(part 1 of 2)
# Autodesk Inventor assembly: #SHOOTER.3
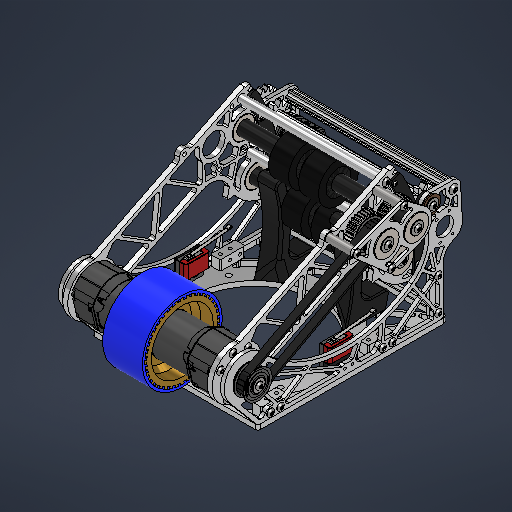
[picture p0: Inventor's stored thumbnail of the model, 512x512]
Saved by Autodesk Inventor 2026.1 (Build 301233020, 233B)
## iProperties
Created: 2026-01-27
Part Number: #SHOOTER.3
Document SubType Name: Assembly
Designer: Owen L
Mass: 5560.26 g
Surface Area: 8956.44 cm^2
Volume: 1678.59 cm^3
Density: 3.31246 g/cm^3
Author: Owen L
## Documents named in this file (55)
- C:\Users\Owen\Documents\GitHub\2026-Robot-Mechanical\Shooter\Shooter - Front Motors\#SHOOTER.FRONT_MOTORS.iam
- C:\Users\Owen\Documents\GitHub\2026-Robot-Mechanical\Shooter\Shooter - Front Motors\PLATE,SHOOTER,SIDE.ipt
- C:\Users\Owen\Documents\GitHub\2026-Robot-Mechanical\#1_CAD Library\Electronics\CONTROLS,SPARK_FLEX.ipt
- C:\Users\Owen\Documents\GitHub\2026-Robot-Mechanical\#1_CAD Library\Power Transmission\Bushings\PURCHASED,BUSHING,13.75mmID,0.75inOD.ipt
- C:\Users\Owen\Documents\GitHub\2026-Robot-Mechanical\#1_CAD Library\Power Transmission\Bearings\PURCHASED,HEX_BEARING.ipt
- C:\Users\Owen\Documents\GitHub\2026-Robot-Mechanical\#1_CAD Library\Motors\MOTOR,REV,NEO,VORTEX.ipt
- C:\Users\Owen\Documents\GitHub\2026-Robot-Mechanical\#1_CAD Library\Motors\MOTOR,REV,NEO,550.ipt
- C:\Users\Owen\Documents\GitHub\2026-Robot-Mechanical\#1_CAD Library\Power Transmission\UltraPlanetary\PURCHASED,REV,ULTRAPLANETARY,2-STAGE.iam
- C:\Users\Owen\Documents\GitHub\2026-Robot-Mechanical\Shooter\Shooter - Front Motors\#SHOOTER.3\Design Accelerator\PLATE,HOOD,SIDE.ipt
- C:\Users\Owen\Documents\GitHub\2026-Robot-Mechanical\Shooter\Shooter - Front Motors\#SHOOTER.3\Design Accelerator\PLATE.HOOD,PINION,GEAR.ipt
- C:\Users\Owen\Documents\GitHub\2026-Robot-Mechanical\Shooter\Shooter - Front Motors\STOCK,HEX,ROUND,HOOD.ipt
- C:\Users\Owen\Documents\GitHub\2026-Robot-Mechanical\#1_CAD Library\Power Transmission\Pulleys\PURCHASED,HTD5mm,20T,PULLEY.ipt
- C:\Users\Owen\Documents\GitHub\2026-Robot-Mechanical\Shooter\Shooter - Front Motors\#SHOOTER.3\Design Accelerator\PLATE,HOOD,DRIVE,GEAR,SHAFT.ipt
- C:\Users\Owen\Documents\GitHub\2026-Robot-Mechanical\Shooter\Shooter - Front Motors\#SHOOTER.3\Design Accelerator\PLATE,HOOD,DRIVE,GEAR,MOTOR.ipt
- C:\Users\Owen\Documents\GitHub\2026-Robot-Mechanical\Shooter\Shooter - Front Motors\STOCK,SHAFT,HEX,SHOOTER.ipt
- C:\Users\Owen\Documents\GitHub\2026-Robot-Mechanical\Shooter\Shooter - Front Motors\#SHOOTER.3\PURCHASED,10-32,0.375inOD,STANDOFF.ipt
- C:\Users\Owen\Documents\GitHub\2026-Robot-Mechanical\Shooter\Shooter - Front Motors\PLATE,BEARING,MOUNT.ipt
- C:\Users\Owen\Documents\GitHub\2026-Robot-Mechanical\Shooter\Shooter - Front Motors\STOCK,SHAFT,HEX,HOOD,WHEELS,LONG.ipt
- C:\Users\Owen\Documents\GitHub\2026-Robot-Mechanical\Shooter\Shooter - Front Motors\STOCK,SHAFT,HEX,HOOD,REVERSER.ipt
- C:\Users\Owen\Documents\GitHub\2026-Robot-Mechanical\Shooter\Shooter - Front Motors\STOCK,SHAFT,HEX,HOOD,WHEELS,SHORT.ipt
- C:\Users\Owen\Documents\GitHub\2026-Robot-Mechanical\Shooter\Shooter - Front Motors\PLATE,SHOOTER,BOTTOM.ipt
- C:\Users\Owen\Documents\GitHub\2026-Robot-Mechanical\Shooter\Shooter - Front Motors\PLATE,SHOOTER,BACK.ipt
- C:\Users\Owen\Documents\GitHub\2026-Robot-Mechanical\Shooter\Shooter - Front Motors\STOCK,CHURRO,HEX,BACK.ipt
- C:\Users\Owen\Documents\GitHub\2026-Robot-Mechanical\Shooter\Shooter - Front Motors\PURCHASED,WASHER.ipt
- C:\Users\Owen\Documents\GitHub\2026-Robot-Mechanical\#1_CAD Library\Wheels\Shooter\PURCHASED,2inOD,HEX,SHOOTER,WHEEL.ipt
- C:\Users\Owen\Documents\GitHub\2026-Robot-Mechanical\#1_CAD Library\Building Materials\Fasteners\Bolts\PURCHASED,0.25-20x0.5in,BUTTONHEAD,BOLT.ipt
- C:\Users\Owen\Documents\GitHub\2026-Robot-Mechanical\#1_CAD Library\Building Materials\Fasteners\Bolts\PURCHASED,10-32x0.5in,BUTTONHEAD,BOLT.ipt
- C:\Users\Owen\Documents\GitHub\2026-Robot-Mechanical\#1_CAD Library\Building Materials\Fasteners\Bolts\PURCHASED,M3x10mm,BUTTONHEAD,BOLT.ipt
- C:\Users\Owen\Documents\GitHub\2026-Robot-Mechanical\Shooter\Shooter - Front Motors\3DPRINT,HOOD,DRIVEGEAR,SPACER.ipt
- C:\Users\Owen\Documents\GitHub\2026-Robot-Mechanical\Shooter\Shooter - Front Motors\3DPRINT,REVERSERGEAR,SPACER.ipt
- C:\Users\Owen\Documents\GitHub\2026-Robot-Mechanical\Shooter\Shooter - Front Motors\3DPRINT,BACKROLLERS,OPENSIDE,SPACER.ipt
- C:\Users\Owen\Documents\GitHub\2026-Robot-Mechanical\Shooter\Shooter - Front Motors\3DPRINT,BACKROLLERS,PULLEYSIDE,SPACER.ipt
- C:\Users\Owen\Documents\GitHub\2026-Robot-Mechanical\Shooter\Shooter - Front Motors\3DPRINT,BACKROLLERS,INTERROLLER,SPACER.ipt
- C:\Users\Owen\Documents\GitHub\2026-Robot-Mechanical\#1_CAD Library\Power Transmission\Gears\PURCHASED,GEAR,20DP,30T,HEX.ipt
- C:\Users\Owen\Documents\GitHub\2026-Robot-Mechanical\Shooter\Shooter - Front Motors\3DPRINT,BACKRAIL.ipt
- C:\Users\Owen\Documents\GitHub\2026-Robot-Mechanical\Shooter\Shooter - Front Motors\3DPRINT,BACKRAIL_MIR.ipt
- C:\Users\Owen\Documents\GitHub\2026-Robot-Mechanical\Shooter\Shooter - Front Motors\PLATE,NUTBLOCK.ipt
- C:\Users\Owen\Documents\GitHub\2026-Robot-Mechanical\#1_CAD Library\Building Materials\Fasteners\Bolts\PURCHASED,M4x12mm,BUTTONHEAD,BOLT.ipt
- C:\Users\Owen\Documents\GitHub\2026-Robot-Mechanical\Shooter\Shooter - Front Motors\STANDIN,45T,HTD5mm,BELT.ipt
- C:\Users\Owen\Documents\GitHub\2026-Robot-Mechanical\Shooter\Shooter - Front Motors\STANDIN,90T,HTD5mm,BELT.ipt
- C:\Users\Owen\Documents\GitHub\2026-Robot-Mechanical\Shooter\Shooter - Front Motors\3DPRINT,FLYWHEELTOHOOD,SPACER.ipt
- C:\Users\Owen\Documents\GitHub\2026-Robot-Mechanical\Shooter\Shooter - Front Motors\STOCK,HOOD,SPACER,10-32,6.25in.ipt
- C:\Users\Owen\Documents\GitHub\2026-Robot-Mechanical\Shooter\Shooter - Front Motors\3DPRINT,SIDEPLATETOHOOD,SPACER .ipt
- C:\Users\Owen\Documents\GitHub\2026-Robot-Mechanical\Shooter\Shooter - Front Motors\3DPRINT,SIDEPLATETOHOODGEAR,SPACER.ipt
- C:\Users\Owen\Documents\GitHub\2026-Robot-Mechanical\Shooter\Shooter - Front Motors\3DPRINT,BUSHINGTOHOODDRIVEGEAR,SPACER.ipt
- C:\Users\Owen\Documents\GitHub\2026-Robot-Mechanical\Shooter\Shooter - Front Motors\3DPRINT,HOOD,ALIGNMENT,PLATES.ipt
- C:\Users\Owen\Documents\GitHub\2026-Robot-Mechanical\#1_CAD Library\Building Materials\Fasteners\Bolts\PURCHASED,M3x16mm,BUTTONHEAD,BOLT.ipt
- C:\Users\Owen\Documents\GitHub\2026-Robot-Mechanical\#1_CAD Library\Building Materials\Fasteners\Nuts\PURCHASED,M3,NYLOCK,NUT.ipt
- C:\Users\Owen\Documents\GitHub\2026-Robot-Mechanical\#1_CAD Library\Electronics\CONTROLS,LIMIT_SWITCH,VEX.iam
- C:\Users\Owen\Documents\GitHub\2026-Robot-Mechanical\Shooter\Shooter - Front Motors\3DPRINT,LIMIT_SWITCH,SPACER.ipt
- C:\Users\Owen\Documents\GitHub\2026-Robot-Mechanical\Shooter\Shooter - Front Motors\3DPRINT,LIMIT_SWITCH,SPACER,RIGHT.ipt
- C:\Users\Owen\Documents\GitHub\2026-Robot-Mechanical\Shooter\Shooter - Front Motors\PLATE,FLYWHEEL,HUB.ipt
- C:\Users\Owen\Documents\GitHub\2026-Robot-Mechanical\Shooter\Shooter - Front Motors\CAST,FLYWHEEL,GRIP.ipt
- C:\Users\Owen\Documents\GitHub\2026-Robot-Mechanical\#1_CAD Library\Electronics\CONTROLS,SPARK_MAX.ipt
- C:\Users\Owen\Documents\GitHub\2026-Robot-Mechanical\Shooter\Shooter - Front Motors\3DPRINT,SPARK_MAX,MOUNT.ipt
## Components (192 placed, 54 different names)
1. PLATE,SHOOTER,SIDE:1 — Insert:2, Mate:2, Insert:3, Insert:4, Mate:6, Mate:36, Insert:82, Insert:83, Insert:84, Insert:85, Mate:120, Insert:110, Insert:111, Insert:112, Insert:113, Insert:114, Insert:146, Mate:182, Mate:187, Mate:189, Insert:195, Insert:196
2. CONTROLS,SPARK_FLEX:1 — Mate:3, Mate:4, Mate:5, Insert:188, Insert:189
3. CONTROLS,SPARK_FLEX:2 — Mate:12, Mate:13, Mate:14, Insert:190, Insert:191
4. PURCHASED,BUSHING,13.75mmID,0.75inOD:1 — Insert:3, Mate:8, Mate:166, Mate:173
5. PURCHASED,BUSHING,13.75mmID,0.75inOD:2 — Insert:7, Mate:11, Mate:170
6. PURCHASED,HEX_BEARING:1 — Insert:4, Mate:30, Mate:31, Mate:191, Mate:192
7. MOTOR,REV,NEO,VORTEX:1 — Mate:3, Mate:4, Mate:5
8. MOTOR,REV,NEO,VORTEX:2 — Mate:12, Mate:13, Mate:14, Mate:209
9. MOTOR,REV,NEO,550:1 — Insert:1, Mate:1
10. PURCHASED,REV,ULTRAPLANETARY,2-STAGE:1 [sub-assembly] — Insert:1, Mate:1, Insert:2, Mate:2, Flush:1, Insert:14, Mate:26
11. PLATE,HOOD,SIDE:1 — Mate:6, Mate:7, Mate:15, Insert:15, Insert:16, Mate:27, Insert:20, Symmetry:1, Insert:152, Insert:154, Insert:155, Mate:174, Insert:161, Insert:163, Insert:164, Insert:165, Insert:188, Insert:189, Insert:205, Insert:206, Insert:207, Insert:208, Insert:209, Insert:210
12. PLATE.HOOD,PINION,GEAR:1 — Mate:22, Mate:23, Mate:163, Mate:167
13. PLATE,HOOD,SIDE:2 — Mate:7, Mate:15, Insert:17, Insert:18, Mate:27, Insert:21, Insert:24, Insert:25, Insert:26, Insert:31, Insert:91, Insert:92, Insert:93, Symmetry:1, Mate:147, Mate:148, Mate:150, Insert:153, Insert:156, Insert:157, Insert:166, Insert:167, Insert:168, Insert:169, Insert:190, Insert:191, Insert:199, Insert:200, Insert:201, Insert:202, Insert:203, Insert:204
14. STOCK,HEX,ROUND,HOOD:1 — Mate:8, Flush:1, Mate:11, Mate:20, Mate:21, Mate:22, Mate:23, Mate:24, Mate:25, Insert:47, Insert:55, Mate:83, Mate:84, Mate:164, Mate:165, Mate:168, Mate:169, Mate:171, Mate:172
15. PURCHASED,HTD5mm,20T,PULLEY:1 — Mate:59, Mate:60, Mate:64, Mate:97, Mate:152
16. PLATE,SHOOTER,SIDE:2 — Insert:7, Insert:19, Mate:36, Insert:40, Insert:101, Insert:104, Insert:124, Insert:125, Insert:126, Insert:127, Insert:145, Mate:149, Insert:192, Insert:193, Insert:197, Insert:198, Mate:196, Mate:197, Mate:201, Mate:202
17. PLATE.HOOD,PINION,GEAR:2 — Mate:20, Mate:21, Mate:85
18. PLATE,HOOD,DRIVE,GEAR,SHAFT:1 — Mate:24, Mate:25, Flush:2
19. PLATE,HOOD,DRIVE,GEAR,MOTOR:1 — Insert:14, Mate:26, Flush:2, Insert:77, Insert:78, Insert:79, Insert:80, Insert:81
20. PURCHASED,HEX_BEARING:5 — Insert:15, Mate:37, Mate:38, Flush:3, Mate:194
21. PURCHASED,HEX_BEARING:6 — Insert:16, Mate:39, Mate:40, Flush:4
22. PURCHASED,HEX_BEARING:7 — Insert:17, Mate:64, Mate:128
23. PURCHASED,HEX_BEARING:8 — Insert:18, Mate:63
24. STOCK,SHAFT,HEX,SHOOTER:1 — Mate:30, Mate:31, Insert:50, Insert:51, Mate:141, Mate:142, Flush:9, Mate:153, Mate:154, Mate:157, Mate:158, Mate:160, Mate:161, Mate:207, Mate:208, Rotation:4
25. PURCHASED,HEX_BEARING:9 — Insert:19, Mate:155
26. PURCHASED,HEX_BEARING:10 — Insert:20, Mate:162
27. PURCHASED,HEX_BEARING:11 — Insert:21, Mate:159
28. PURCHASED,HEX_BEARING:12 — Insert:31, Mate:41, Mate:42, Flush:5, Mate:129
29. PURCHASED,10-32,0.375inOD,STANDOFF:1 — Insert:24, Insert:97
30. PURCHASED,10-32,0.375inOD,STANDOFF:2 — Insert:25
31. PURCHASED,10-32,0.375inOD,STANDOFF:3 — Insert:26
32. PLATE,BEARING,MOUNT:1 — Insert:94, Insert:96, Insert:97, Insert:98, Insert:99, Insert:100
33. PURCHASED,HEX_BEARING:14 — Mate:88, Mate:121, Mate:122, Insert:96
34. PURCHASED,HEX_BEARING:15 — Insert:94, Mate:123
35. STOCK,SHAFT,HEX,HOOD,WHEELS,LONG:1 — Mate:37, Mate:38, Flush:3, Mate:59, Mate:60, Insert:48, Insert:53, Mate:65, Mate:66, Mate:67, Mate:68, Mate:86, Mate:87, Mate:89, Mate:90, Mate:95, Mate:96, Mate:101, Mate:102, Mate:121, Mate:122, Mate:126, Mate:127, Rotation:1, Rotation:2, Rotation:3
36. STOCK,SHAFT,HEX,HOOD,REVERSER:1 — Mate:41, Mate:42, Flush:5, Insert:52, Insert:86, Mate:123, Mate:124, Mate:125, Mate:144, Mate:145, Rotation:1, Rotation:2, Rotation:4
37. STOCK,SHAFT,HEX,HOOD,WHEELS,SHORT:1 — Mate:39, Mate:40, Flush:4, Mate:61, Mate:62, Insert:49, Insert:54, Mate:69, Mate:70, Mate:71, Mate:72, Mate:92, Mate:93, Mate:98, Mate:99, Mate:104, Mate:105, Rotation:3
38. PLATE,SHOOTER,BOTTOM:1 — Mate:120, Mate:131, Insert:102, Insert:103, Insert:107, Insert:115, Insert:116, Insert:117, Insert:118, Insert:119, Insert:120, Insert:121, Insert:122, Insert:137, Insert:138, Insert:139, Insert:140, Insert:141, Insert:142, Insert:143, Insert:144, Insert:151, Mate:137, Insert:158, Mate:174, Mate:183, Mate:185, Mate:193, Insert:211, Mate:210, Mate:211, Mate:213
39. PLATE,SHOOTER,BACK:1 — Insert:128, Insert:129, Insert:192, Insert:193, Insert:194, Mate:195, Mate:216, Mate:217, Mate:218, Mate:219
40. PURCHASED,HTD5mm,20T,PULLEY:2 — Mate:61, Mate:62, Mate:63, Mate:100
41. STOCK,CHURRO,HEX,BACK:1 — Insert:40
42. PURCHASED,2inOD,HEX,SHOOTER,WHEEL:1 — Mate:65, Mate:66, Mate:73, Mate:103
43. PURCHASED,2inOD,HEX,SHOOTER,WHEEL:2 — Mate:67, Mate:68, Mate:73, Flush:8, Mate:91
44. PURCHASED,2inOD,HEX,SHOOTER,WHEEL:3 — Mate:69, Mate:70, Mate:74, Mate:106
45. PURCHASED,2inOD,HEX,SHOOTER,WHEEL:4 — Mate:71, Mate:72, Mate:74, Flush:8, Mate:94
46. PURCHASED,0.25-20x0.5in,BUTTONHEAD,BOLT:1 — Insert:146
47. PURCHASED,0.25-20x0.5in,BUTTONHEAD,BOLT:4 — Insert:145
48. PURCHASED,M3x10mm,BUTTONHEAD,BOLT:1 — Insert:77
49. PURCHASED,WASHER:2 — Insert:47, Insert:62
50. PURCHASED,WASHER:3 — Insert:48, Insert:64
51. PURCHASED,WASHER:4 — Insert:49, Insert:63
52. PURCHASED,WASHER:5 — Insert:50, Insert:65, Mate:191
53. PURCHASED,WASHER:6 — Insert:51, Insert:66
54. PURCHASED,WASHER:7 — Insert:52, Insert:67
55. PURCHASED,WASHER:8 — Insert:53, Insert:68
56. PURCHASED,WASHER:9 — Insert:54, Insert:69
57. PURCHASED,WASHER:10 — Insert:55, Insert:70
58. PURCHASED,10-32x0.5in,BUTTONHEAD,BOLT:6 — Insert:62
59. PURCHASED,10-32x0.5in,BUTTONHEAD,BOLT:7 — Insert:63
60. PURCHASED,10-32x0.5in,BUTTONHEAD,BOLT:8 — Insert:65
61. PURCHASED,10-32x0.5in,BUTTONHEAD,BOLT:9 — Insert:64
62. PURCHASED,10-32x0.5in,BUTTONHEAD,BOLT:10 — Insert:66
63. PURCHASED,10-32x0.5in,BUTTONHEAD,BOLT:11 — Insert:67
64. PURCHASED,10-32x0.5in,BUTTONHEAD,BOLT:12 — Insert:68
65. PURCHASED,10-32x0.5in,BUTTONHEAD,BOLT:13 — Insert:69
66. PURCHASED,10-32x0.5in,BUTTONHEAD,BOLT:14 — Insert:70
67. PURCHASED,10-32x0.5in,BUTTONHEAD,BOLT:16 — Insert:87
68. PURCHASED,M3x10mm,BUTTONHEAD,BOLT:2 — Insert:78
69. PURCHASED,M3x10mm,BUTTONHEAD,BOLT:3 — Insert:80
70. PURCHASED,M3x10mm,BUTTONHEAD,BOLT:4 — Insert:79
71. PURCHASED,M3x10mm,BUTTONHEAD,BOLT:5 — Insert:81
72. PURCHASED,M3x10mm,BUTTONHEAD,BOLT:6 — Insert:82
73. PURCHASED,M3x10mm,BUTTONHEAD,BOLT:7 — Insert:83
74. PURCHASED,M3x10mm,BUTTONHEAD,BOLT:8 — Insert:84
75. PURCHASED,M3x10mm,BUTTONHEAD,BOLT:9 — Insert:85
76. 3DPRINT,HOOD,DRIVEGEAR,SPACER:1 — Mate:83, Mate:84, Mate:85, Mate:163
77. 3DPRINT,REVERSERGEAR,SPACER:1 — Mate:86, Mate:87, Mate:88
78. 3DPRINT,BACKROLLERS,OPENSIDE,SPACER:1 — Mate:89, Mate:90, Mate:91, Mate:194
79. 3DPRINT,BACKROLLERS,OPENSIDE,SPACER:2 — Mate:92, Mate:93, Mate:94
80. 3DPRINT,BACKROLLERS,PULLEYSIDE,SPACER:1 — Mate:95, Mate:96, Mate:97
81. 3DPRINT,BACKROLLERS,PULLEYSIDE,SPACER:2 — Mate:98, Mate:99, Mate:100
82. 3DPRINT,BACKROLLERS,INTERROLLER,SPACER:1 — Mate:101, Mate:102, Mate:103
83. 3DPRINT,BACKROLLERS,INTERROLLER,SPACER:2 — Mate:104, Mate:105, Mate:106
84. PURCHASED,WASHER:12 — Insert:86, Insert:87
85. PURCHASED,10-32x0.5in,BUTTONHEAD,BOLT:21 — Insert:99
86. PURCHASED,10-32x0.5in,BUTTONHEAD,BOLT:22 — Insert:98
87. PURCHASED,10-32x0.5in,BUTTONHEAD,BOLT:23 — Insert:100
88. PURCHASED,10-32x0.5in,BUTTONHEAD,BOLT:24 — Insert:91
89. PURCHASED,10-32x0.5in,BUTTONHEAD,BOLT:25 — Insert:92
90. PURCHASED,10-32x0.5in,BUTTONHEAD,BOLT:26 — Insert:93
91. PURCHASED,GEAR,20DP,30T,HEX:1 — Mate:124, Mate:125, Mate:129, Mate:146
92. PURCHASED,GEAR,20DP,30T,HEX:2 — Mate:126, Mate:127, Mate:128
93. 3DPRINT,BACKRAIL:1 — Mate:131, Insert:158, Mate:212
94. 3DPRINT,BACKRAIL_MIR:1 — Insert:151, Mate:137
95. PLATE,NUTBLOCK:1 — Insert:101, Insert:102
96. PLATE,NUTBLOCK:2 — Insert:103, Insert:104
97. PLATE,NUTBLOCK:4 — Insert:107, Mate:181
98. PLATE,NUTBLOCK:5 — Insert:110, Mate:193
99. PURCHASED,10-32x0.5in,BUTTONHEAD,BOLT:27 — Insert:114
100. PURCHASED,10-32x0.5in,BUTTONHEAD,BOLT:28 — Insert:113
101. PURCHASED,10-32x0.5in,BUTTONHEAD,BOLT:29 — Insert:112
102. PURCHASED,10-32x0.5in,BUTTONHEAD,BOLT:30 — Insert:111
103. PURCHASED,10-32x0.5in,BUTTONHEAD,BOLT:31 — Insert:115
104. PURCHASED,10-32x0.5in,BUTTONHEAD,BOLT:32 — Insert:116
105. PURCHASED,10-32x0.5in,BUTTONHEAD,BOLT:33 — Insert:117
106. PURCHASED,10-32x0.5in,BUTTONHEAD,BOLT:34 — Insert:118
107. PURCHASED,10-32x0.5in,BUTTONHEAD,BOLT:35 — Insert:119
108. PURCHASED,10-32x0.5in,BUTTONHEAD,BOLT:36 — Insert:120
109. PURCHASED,10-32x0.5in,BUTTONHEAD,BOLT:37 — Insert:121
110. PURCHASED,10-32x0.5in,BUTTONHEAD,BOLT:38 — Insert:122
111. PURCHASED,10-32x0.5in,BUTTONHEAD,BOLT:39 — Insert:211
112. PURCHASED,10-32x0.5in,BUTTONHEAD,BOLT:40 — Insert:124
113. PURCHASED,10-32x0.5in,BUTTONHEAD,BOLT:41 — Insert:125
114. PURCHASED,10-32x0.5in,BUTTONHEAD,BOLT:42 — Insert:126
115. PURCHASED,10-32x0.5in,BUTTONHEAD,BOLT:43 — Insert:127
116. PURCHASED,10-32x0.5in,BUTTONHEAD,BOLT:44 — Insert:128
117. PURCHASED,10-32x0.5in,BUTTONHEAD,BOLT:45 — Insert:129
118. PURCHASED,M4x12mm,BUTTONHEAD,BOLT:1 — Insert:137
119. PURCHASED,M4x12mm,BUTTONHEAD,BOLT:2 — Insert:138, Mate:212
120. PURCHASED,M4x12mm,BUTTONHEAD,BOLT:3 — Insert:139
121. PURCHASED,M4x12mm,BUTTONHEAD,BOLT:4 — Insert:140
122. PURCHASED,M4x12mm,BUTTONHEAD,BOLT:5 — Insert:141
123. PURCHASED,M4x12mm,BUTTONHEAD,BOLT:6 — Insert:142
124. PURCHASED,M4x12mm,BUTTONHEAD,BOLT:7 — Insert:143
125. PURCHASED,M4x12mm,BUTTONHEAD,BOLT:8 — Insert:144
126. PURCHASED,HTD5mm,20T,PULLEY:3 — Mate:141, Mate:142, Flush:9
127. PURCHASED,HTD5mm,20T,PULLEY:4 — Mate:144, Mate:145, Mate:146, Mate:151
128. STANDIN,45T,HTD5mm,BELT:1 — Mate:147, Mate:148, Mate:152
129. STANDIN,90T,HTD5mm,BELT:1 — Mate:149, Mate:150, Mate:151
130. 3DPRINT,FLYWHEELTOHOOD,SPACER:1 — Mate:153, Mate:154, Mate:155
131. STOCK,HOOD,SPACER,10-32,6.25in:1 — Insert:152
132. STOCK,HOOD,SPACER,10-32,6.25in:2 — Insert:153
133. PURCHASED,10-32x0.5in,BUTTONHEAD,BOLT:49 — Insert:154
134. PURCHASED,10-32x0.5in,BUTTONHEAD,BOLT:50 — Insert:156
135. PURCHASED,10-32x0.5in,BUTTONHEAD,BOLT:51 — Insert:155
136. PURCHASED,10-32x0.5in,BUTTONHEAD,BOLT:52 — Insert:157
137. 3DPRINT,SIDEPLATETOHOOD,SPACER :1 — Mate:157, Mate:158, Mate:159
138. 3DPRINT,SIDEPLATETOHOODGEAR,SPACER:1 — Mate:171, Mate:172, Mate:173
139. 3DPRINT,BUSHINGTOHOODDRIVEGEAR,SPACER:1 — Mate:164, Mate:165, Mate:166, Mate:167
140. 3DPRINT,SIDEPLATETOHOOD,SPACER :2 — Mate:160, Mate:161, Mate:162, Mate:192
141. 3DPRINT,BUSHINGTOHOODDRIVEGEAR,SPACER:2 — Mate:168, Mate:169, Mate:170
142. 3DPRINT,HOOD,ALIGNMENT,PLATES:1 — Insert:161, Insert:165, Insert:174, Insert:175, Insert:176, Insert:177, Insert:178
143. 3DPRINT,HOOD,ALIGNMENT,PLATES:2 — Insert:163, Insert:164, Insert:179, Insert:180, Insert:181, Insert:182, Insert:183
144. 3DPRINT,HOOD,ALIGNMENT,PLATES:3 — Insert:166, Insert:167, Insert:170, Insert:171, Insert:172, Insert:173
145. 3DPRINT,HOOD,ALIGNMENT,PLATES:4 — Insert:168, Insert:169, Insert:184, Insert:185, Insert:186, Insert:187
146. PURCHASED,M3x16mm,BUTTONHEAD,BOLT:1 — Insert:170
147. PURCHASED,M3x16mm,BUTTONHEAD,BOLT:2 — Insert:171
148. PURCHASED,M3x16mm,BUTTONHEAD,BOLT:3 — Insert:172
149. PURCHASED,M3x16mm,BUTTONHEAD,BOLT:4 — Insert:173
150. PURCHASED,M3x16mm,BUTTONHEAD,BOLT:5 — Insert:174
151. PURCHASED,M3x16mm,BUTTONHEAD,BOLT:6 — Insert:175
152. PURCHASED,M3x16mm,BUTTONHEAD,BOLT:7 — Insert:176
153. PURCHASED,M3x16mm,BUTTONHEAD,BOLT:8 — Insert:177
154. PURCHASED,M3x16mm,BUTTONHEAD,BOLT:9 — Insert:178
155. PURCHASED,M3,NYLOCK,NUT:1 — Insert:186
156. PURCHASED,M3,NYLOCK,NUT:3 — Insert:187
157. PURCHASED,M3,NYLOCK,NUT:5 — Insert:185
158. PURCHASED,M3,NYLOCK,NUT:6 — Insert:184
159. PURCHASED,M3,NYLOCK,NUT:7 — Insert:183
160. PURCHASED,M3,NYLOCK,NUT:8 — Insert:182
161. PURCHASED,M3,NYLOCK,NUT:9 — Insert:181
162. PURCHASED,M3,NYLOCK,NUT:10 — Insert:180
163. PURCHASED,M3,NYLOCK,NUT:11 — Insert:179
164. CONTROLS,LIMIT_SWITCH,VEX:1 [sub-assembly] — Mate:184, Mate:185, Mate:186, Mate:188, Mate:190
165. 3DPRINT,LIMIT_SWITCH,SPACER:1 — Mate:181, Mate:182, Mate:183, Mate:184, Mate:186, Flush:10
166. PURCHASED,M4x12mm,BUTTONHEAD,BOLT:9 — Mate:187, Mate:188
167. PURCHASED,M4x12mm,BUTTONHEAD,BOLT:10 — Mate:189, Mate:190
168. PLATE,NUTBLOCK:6 — Insert:194, Mate:195
169. PURCHASED,10-32x0.5in,BUTTONHEAD,BOLT:53 — Insert:195
170. PURCHASED,10-32x0.5in,BUTTONHEAD,BOLT:54 — Insert:196
171. PURCHASED,10-32x0.5in,BUTTONHEAD,BOLT:55 — Insert:197
172. PURCHASED,10-32x0.5in,BUTTONHEAD,BOLT:56 — Insert:198
173. PURCHASED,10-32x0.5in,BUTTONHEAD,BOLT:57 — Insert:201
174. PURCHASED,10-32x0.5in,BUTTONHEAD,BOLT:58 — Insert:200
175. PURCHASED,10-32x0.5in,BUTTONHEAD,BOLT:59 — Insert:199
176. PURCHASED,10-32x0.5in,BUTTONHEAD,BOLT:60 — Insert:203
177. PURCHASED,10-32x0.5in,BUTTONHEAD,BOLT:61 — Insert:204
178. PURCHASED,10-32x0.5in,BUTTONHEAD,BOLT:62 — Insert:202
179. PURCHASED,10-32x0.5in,BUTTONHEAD,BOLT:63 — Insert:205
180. PURCHASED,10-32x0.5in,BUTTONHEAD,BOLT:64 — Insert:207
181. PURCHASED,10-32x0.5in,BUTTONHEAD,BOLT:65 — Insert:208
182. PURCHASED,10-32x0.5in,BUTTONHEAD,BOLT:66 — Insert:206
183. PURCHASED,10-32x0.5in,BUTTONHEAD,BOLT:67 — Insert:210
184. PURCHASED,10-32x0.5in,BUTTONHEAD,BOLT:68 — Insert:209
185. 3DPRINT,LIMIT_SWITCH,SPACER,RIGHT:1 — Mate:196, Mate:197, Mate:198, Mate:199, Mate:200, Flush:10
186. CONTROLS,LIMIT_SWITCH,VEX:2 [sub-assembly] — Mate:198, Mate:199, Mate:200, Mate:203, Mate:204
187. PURCHASED,M4x12mm,BUTTONHEAD,BOLT:11 — Mate:201, Mate:204
188. PURCHASED,M4x12mm,BUTTONHEAD,BOLT:12 — Mate:202, Mate:203
189. PLATE,FLYWHEEL,HUB:1 — Mate:207, Mate:208, Mate:209, Mate:214, Flush:12, Mate:215
190. CAST,FLYWHEEL,GRIP:2 — Mate:214, Flush:12, Mate:215
191. CONTROLS,SPARK_MAX:1 — Mate:216, Mate:220, Mate:221
192. 3DPRINT,SPARK_MAX,MOUNT:1 — Mate:217, Mate:218, Mate:219, Mate:220, Mate:221
## Relationships (315: Mate 153, Insert 148, Flush 9, RelateRotation 4, Symmetry 1)
- Insert:1: MOTOR,REV,NEO,550:1 ↔ PURCHASED,REV,ULTRAPLANETARY,2-STAGE:1
- Mate:1: MOTOR,REV,NEO,550:1 ↔ PURCHASED,REV,ULTRAPLANETARY,2-STAGE:1
- Insert:2: PLATE,SHOOTER,SIDE:1 ↔ PURCHASED,REV,ULTRAPLANETARY,2-STAGE:1
- Mate:2: PLATE,SHOOTER,SIDE:1 ↔ PURCHASED,REV,ULTRAPLANETARY,2-STAGE:1
- Insert:3: PLATE,SHOOTER,SIDE:1 ↔ PURCHASED,BUSHING,13.75mmID,0.75inOD:1
- Insert:4: PLATE,SHOOTER,SIDE:1 ↔ PURCHASED,HEX_BEARING:1
- Mate:3: CONTROLS,SPARK_FLEX:1 ↔ MOTOR,REV,NEO,VORTEX:1
- Mate:4: CONTROLS,SPARK_FLEX:1 ↔ MOTOR,REV,NEO,VORTEX:1
- Mate:5: CONTROLS,SPARK_FLEX:1 ↔ MOTOR,REV,NEO,VORTEX:1
- Mate:6: PLATE,SHOOTER,SIDE:1 ↔ PLATE,HOOD,SIDE:1
- Mate:7 (177.8 mm): PLATE,HOOD,SIDE:1 ↔ PLATE,HOOD,SIDE:2
- Mate:8: PURCHASED,BUSHING,13.75mmID,0.75inOD:1 ↔ STOCK,HEX,ROUND,HOOD:1
- Flush:1 (-6.35 mm): PURCHASED,REV,ULTRAPLANETARY,2-STAGE:1 ↔ STOCK,HEX,ROUND,HOOD:1
- Insert:7: PURCHASED,BUSHING,13.75mmID,0.75inOD:2 ↔ PLATE,SHOOTER,SIDE:2
- Mate:11: PURCHASED,BUSHING,13.75mmID,0.75inOD:2 ↔ STOCK,HEX,ROUND,HOOD:1
- Mate:12: CONTROLS,SPARK_FLEX:2 ↔ MOTOR,REV,NEO,VORTEX:2
- Mate:13: CONTROLS,SPARK_FLEX:2 ↔ MOTOR,REV,NEO,VORTEX:2
- Mate:14: CONTROLS,SPARK_FLEX:2 ↔ MOTOR,REV,NEO,VORTEX:2
- Mate:15: PLATE,HOOD,SIDE:1 ↔ PLATE,HOOD,SIDE:2
- Mate:20: STOCK,HEX,ROUND,HOOD:1 ↔ PLATE.HOOD,PINION,GEAR:2
- Mate:21: STOCK,HEX,ROUND,HOOD:1 ↔ PLATE.HOOD,PINION,GEAR:2
- Mate:22: PLATE.HOOD,PINION,GEAR:1 ↔ STOCK,HEX,ROUND,HOOD:1
- Mate:23: PLATE.HOOD,PINION,GEAR:1 ↔ STOCK,HEX,ROUND,HOOD:1
- Mate:24: STOCK,HEX,ROUND,HOOD:1 ↔ PLATE,HOOD,DRIVE,GEAR,SHAFT:1
- Mate:25: STOCK,HEX,ROUND,HOOD:1 ↔ PLATE,HOOD,DRIVE,GEAR,SHAFT:1
- Insert:14: PURCHASED,REV,ULTRAPLANETARY,2-STAGE:1 ↔ PLATE,HOOD,DRIVE,GEAR,MOTOR:1
- Mate:26: PURCHASED,REV,ULTRAPLANETARY,2-STAGE:1 ↔ PLATE,HOOD,DRIVE,GEAR,MOTOR:1
- Flush:2: PLATE,HOOD,DRIVE,GEAR,SHAFT:1 ↔ PLATE,HOOD,DRIVE,GEAR,MOTOR:1
- Insert:15: PLATE,HOOD,SIDE:1 ↔ PURCHASED,HEX_BEARING:5
- Insert:16: PLATE,HOOD,SIDE:1 ↔ PURCHASED,HEX_BEARING:6
- Insert:17: PLATE,HOOD,SIDE:2 ↔ PURCHASED,HEX_BEARING:7
- Insert:18: PLATE,HOOD,SIDE:2 ↔ PURCHASED,HEX_BEARING:8
- Mate:27: PLATE,HOOD,SIDE:1 ↔ PLATE,HOOD,SIDE:2
- Mate:30: PURCHASED,HEX_BEARING:1 ↔ STOCK,SHAFT,HEX,SHOOTER:1
- Mate:31: PURCHASED,HEX_BEARING:1 ↔ STOCK,SHAFT,HEX,SHOOTER:1
- Insert:19: PLATE,SHOOTER,SIDE:2 ↔ PURCHASED,HEX_BEARING:9
- Insert:20: PLATE,HOOD,SIDE:1 ↔ PURCHASED,HEX_BEARING:10
- Insert:21: PLATE,HOOD,SIDE:2 ↔ PURCHASED,HEX_BEARING:11
- Mate:36: PLATE,SHOOTER,SIDE:1 ↔ PLATE,SHOOTER,SIDE:2
- Insert:24: PLATE,HOOD,SIDE:2 ↔ PURCHASED,10-32,0.375inOD,STANDOFF:1
- Insert:25: PLATE,HOOD,SIDE:2 ↔ PURCHASED,10-32,0.375inOD,STANDOFF:2
- Insert:26: PLATE,HOOD,SIDE:2 ↔ PURCHASED,10-32,0.375inOD,STANDOFF:3
- Mate:37: PURCHASED,HEX_BEARING:5 ↔ STOCK,SHAFT,HEX,HOOD,WHEELS,LONG:1
- Mate:38: PURCHASED,HEX_BEARING:5 ↔ STOCK,SHAFT,HEX,HOOD,WHEELS,LONG:1
- Flush:3: PURCHASED,HEX_BEARING:5 ↔ STOCK,SHAFT,HEX,HOOD,WHEELS,LONG:1
- Insert:31: PLATE,HOOD,SIDE:2 ↔ PURCHASED,HEX_BEARING:12
- Mate:39: PURCHASED,HEX_BEARING:6 ↔ STOCK,SHAFT,HEX,HOOD,WHEELS,SHORT:1
- Mate:40: PURCHASED,HEX_BEARING:6 ↔ STOCK,SHAFT,HEX,HOOD,WHEELS,SHORT:1
- Flush:4: PURCHASED,HEX_BEARING:6 ↔ STOCK,SHAFT,HEX,HOOD,WHEELS,SHORT:1
- Mate:41: PURCHASED,HEX_BEARING:12 ↔ STOCK,SHAFT,HEX,HOOD,REVERSER:1
- Mate:42: PURCHASED,HEX_BEARING:12 ↔ STOCK,SHAFT,HEX,HOOD,REVERSER:1
- Flush:5: PURCHASED,HEX_BEARING:12 ↔ STOCK,SHAFT,HEX,HOOD,REVERSER:1
- Mate:59: PURCHASED,HTD5mm,20T,PULLEY:1 ↔ STOCK,SHAFT,HEX,HOOD,WHEELS,LONG:1
- Mate:60: PURCHASED,HTD5mm,20T,PULLEY:1 ↔ STOCK,SHAFT,HEX,HOOD,WHEELS,LONG:1
- Mate:61: STOCK,SHAFT,HEX,HOOD,WHEELS,SHORT:1 ↔ PURCHASED,HTD5mm,20T,PULLEY:2
- Mate:62: STOCK,SHAFT,HEX,HOOD,WHEELS,SHORT:1 ↔ PURCHASED,HTD5mm,20T,PULLEY:2
- Mate:63: PURCHASED,HEX_BEARING:8 ↔ PURCHASED,HTD5mm,20T,PULLEY:2
- Mate:64: PURCHASED,HTD5mm,20T,PULLEY:1 ↔ PURCHASED,HEX_BEARING:7
- Insert:40: PLATE,SHOOTER,SIDE:2 ↔ STOCK,CHURRO,HEX,BACK:1
- Insert:47: STOCK,HEX,ROUND,HOOD:1 ↔ PURCHASED,WASHER:2
- Insert:48: STOCK,SHAFT,HEX,HOOD,WHEELS,LONG:1 ↔ PURCHASED,WASHER:3
- Insert:49: STOCK,SHAFT,HEX,HOOD,WHEELS,SHORT:1 ↔ PURCHASED,WASHER:4
- Insert:50: STOCK,SHAFT,HEX,SHOOTER:1 ↔ PURCHASED,WASHER:5
- Insert:51: STOCK,SHAFT,HEX,SHOOTER:1 ↔ PURCHASED,WASHER:6
- Insert:52: STOCK,SHAFT,HEX,HOOD,REVERSER:1 ↔ PURCHASED,WASHER:7
- Insert:53: STOCK,SHAFT,HEX,HOOD,WHEELS,LONG:1 ↔ PURCHASED,WASHER:8
- Insert:54: STOCK,SHAFT,HEX,HOOD,WHEELS,SHORT:1 ↔ PURCHASED,WASHER:9
- Insert:55: STOCK,HEX,ROUND,HOOD:1 ↔ PURCHASED,WASHER:10
- Mate:65: STOCK,SHAFT,HEX,HOOD,WHEELS,LONG:1 ↔ PURCHASED,2inOD,HEX,SHOOTER,WHEEL:1
- Mate:66: STOCK,SHAFT,HEX,HOOD,WHEELS,LONG:1 ↔ PURCHASED,2inOD,HEX,SHOOTER,WHEEL:1
- Mate:67: STOCK,SHAFT,HEX,HOOD,WHEELS,LONG:1 ↔ PURCHASED,2inOD,HEX,SHOOTER,WHEEL:2
- Mate:68: STOCK,SHAFT,HEX,HOOD,WHEELS,LONG:1 ↔ PURCHASED,2inOD,HEX,SHOOTER,WHEEL:2
- Mate:69: STOCK,SHAFT,HEX,HOOD,WHEELS,SHORT:1 ↔ PURCHASED,2inOD,HEX,SHOOTER,WHEEL:3
- Mate:70: STOCK,SHAFT,HEX,HOOD,WHEELS,SHORT:1 ↔ PURCHASED,2inOD,HEX,SHOOTER,WHEEL:3
- Mate:71: STOCK,SHAFT,HEX,HOOD,WHEELS,SHORT:1 ↔ PURCHASED,2inOD,HEX,SHOOTER,WHEEL:4
- Mate:72: STOCK,SHAFT,HEX,HOOD,WHEELS,SHORT:1 ↔ PURCHASED,2inOD,HEX,SHOOTER,WHEEL:4
- Mate:73 (12.7 mm): PURCHASED,2inOD,HEX,SHOOTER,WHEEL:1 ↔ PURCHASED,2inOD,HEX,SHOOTER,WHEEL:2
- Mate:74 (12.7 mm): PURCHASED,2inOD,HEX,SHOOTER,WHEEL:3 ↔ PURCHASED,2inOD,HEX,SHOOTER,WHEEL:4
- Insert:62: PURCHASED,WASHER:2 ↔ PURCHASED,10-32x0.5in,BUTTONHEAD,BOLT:6
- Insert:63: PURCHASED,WASHER:4 ↔ PURCHASED,10-32x0.5in,BUTTONHEAD,BOLT:7
- Insert:64: PURCHASED,WASHER:3 ↔ PURCHASED,10-32x0.5in,BUTTONHEAD,BOLT:9
- Insert:65: PURCHASED,WASHER:5 ↔ PURCHASED,10-32x0.5in,BUTTONHEAD,BOLT:8
- Insert:66: PURCHASED,WASHER:6 ↔ PURCHASED,10-32x0.5in,BUTTONHEAD,BOLT:10
- Insert:67: PURCHASED,WASHER:7 ↔ PURCHASED,10-32x0.5in,BUTTONHEAD,BOLT:11
- Insert:68: PURCHASED,WASHER:8 ↔ PURCHASED,10-32x0.5in,BUTTONHEAD,BOLT:12
- Insert:69: PURCHASED,WASHER:9 ↔ PURCHASED,10-32x0.5in,BUTTONHEAD,BOLT:13
- Insert:70: PURCHASED,WASHER:10 ↔ PURCHASED,10-32x0.5in,BUTTONHEAD,BOLT:14
- Insert:77: PLATE,HOOD,DRIVE,GEAR,MOTOR:1 ↔ PURCHASED,M3x10mm,BUTTONHEAD,BOLT:1
- Insert:78: PLATE,HOOD,DRIVE,GEAR,MOTOR:1 ↔ PURCHASED,M3x10mm,BUTTONHEAD,BOLT:2
- Insert:79: PLATE,HOOD,DRIVE,GEAR,MOTOR:1 ↔ PURCHASED,M3x10mm,BUTTONHEAD,BOLT:4
- Insert:80: PLATE,HOOD,DRIVE,GEAR,MOTOR:1 ↔ PURCHASED,M3x10mm,BUTTONHEAD,BOLT:3
- Insert:81: PLATE,HOOD,DRIVE,GEAR,MOTOR:1 ↔ PURCHASED,M3x10mm,BUTTONHEAD,BOLT:5
- Insert:82: PLATE,SHOOTER,SIDE:1 ↔ PURCHASED,M3x10mm,BUTTONHEAD,BOLT:6
- Insert:83: PLATE,SHOOTER,SIDE:1 ↔ PURCHASED,M3x10mm,BUTTONHEAD,BOLT:7
- Insert:84: PLATE,SHOOTER,SIDE:1 ↔ PURCHASED,M3x10mm,BUTTONHEAD,BOLT:8
- Insert:85: PLATE,SHOOTER,SIDE:1 ↔ PURCHASED,M3x10mm,BUTTONHEAD,BOLT:9
- Flush:8: PURCHASED,2inOD,HEX,SHOOTER,WHEEL:2 ↔ PURCHASED,2inOD,HEX,SHOOTER,WHEEL:4
- Mate:83: STOCK,HEX,ROUND,HOOD:1 ↔ 3DPRINT,HOOD,DRIVEGEAR,SPACER:1
- Mate:84: STOCK,HEX,ROUND,HOOD:1 ↔ 3DPRINT,HOOD,DRIVEGEAR,SPACER:1
- Mate:85: PLATE.HOOD,PINION,GEAR:2 ↔ 3DPRINT,HOOD,DRIVEGEAR,SPACER:1
- Mate:86: STOCK,SHAFT,HEX,HOOD,WHEELS,LONG:1 ↔ 3DPRINT,REVERSERGEAR,SPACER:1
- Mate:87: STOCK,SHAFT,HEX,HOOD,WHEELS,LONG:1 ↔ 3DPRINT,REVERSERGEAR,SPACER:1
- Mate:88: PURCHASED,HEX_BEARING:14 ↔ 3DPRINT,REVERSERGEAR,SPACER:1
- Mate:89: STOCK,SHAFT,HEX,HOOD,WHEELS,LONG:1 ↔ 3DPRINT,BACKROLLERS,OPENSIDE,SPACER:1
- Mate:90: STOCK,SHAFT,HEX,HOOD,WHEELS,LONG:1 ↔ 3DPRINT,BACKROLLERS,OPENSIDE,SPACER:1
- Mate:91: PURCHASED,2inOD,HEX,SHOOTER,WHEEL:2 ↔ 3DPRINT,BACKROLLERS,OPENSIDE,SPACER:1
- Mate:92: STOCK,SHAFT,HEX,HOOD,WHEELS,SHORT:1 ↔ 3DPRINT,BACKROLLERS,OPENSIDE,SPACER:2
- Mate:93: STOCK,SHAFT,HEX,HOOD,WHEELS,SHORT:1 ↔ 3DPRINT,BACKROLLERS,OPENSIDE,SPACER:2
- Mate:94: PURCHASED,2inOD,HEX,SHOOTER,WHEEL:4 ↔ 3DPRINT,BACKROLLERS,OPENSIDE,SPACER:2
- Mate:95: STOCK,SHAFT,HEX,HOOD,WHEELS,LONG:1 ↔ 3DPRINT,BACKROLLERS,PULLEYSIDE,SPACER:1
- Mate:96: STOCK,SHAFT,HEX,HOOD,WHEELS,LONG:1 ↔ 3DPRINT,BACKROLLERS,PULLEYSIDE,SPACER:1
- Mate:97: PURCHASED,HTD5mm,20T,PULLEY:1 ↔ 3DPRINT,BACKROLLERS,PULLEYSIDE,SPACER:1
- Mate:98: STOCK,SHAFT,HEX,HOOD,WHEELS,SHORT:1 ↔ 3DPRINT,BACKROLLERS,PULLEYSIDE,SPACER:2
- Mate:99: STOCK,SHAFT,HEX,HOOD,WHEELS,SHORT:1 ↔ 3DPRINT,BACKROLLERS,PULLEYSIDE,SPACER:2
- Mate:100: PURCHASED,HTD5mm,20T,PULLEY:2 ↔ 3DPRINT,BACKROLLERS,PULLEYSIDE,SPACER:2
- Mate:101: STOCK,SHAFT,HEX,HOOD,WHEELS,LONG:1 ↔ 3DPRINT,BACKROLLERS,INTERROLLER,SPACER:1
- Mate:102: STOCK,SHAFT,HEX,HOOD,WHEELS,LONG:1 ↔ 3DPRINT,BACKROLLERS,INTERROLLER,SPACER:1
- Mate:103: PURCHASED,2inOD,HEX,SHOOTER,WHEEL:1 ↔ 3DPRINT,BACKROLLERS,INTERROLLER,SPACER:1
- Mate:104: STOCK,SHAFT,HEX,HOOD,WHEELS,SHORT:1 ↔ 3DPRINT,BACKROLLERS,INTERROLLER,SPACER:2
- Mate:105: STOCK,SHAFT,HEX,HOOD,WHEELS,SHORT:1 ↔ 3DPRINT,BACKROLLERS,INTERROLLER,SPACER:2
- Mate:106: PURCHASED,2inOD,HEX,SHOOTER,WHEEL:3 ↔ 3DPRINT,BACKROLLERS,INTERROLLER,SPACER:2
- Insert:86: STOCK,SHAFT,HEX,HOOD,REVERSER:1 ↔ PURCHASED,WASHER:12
- Insert:87: PURCHASED,10-32x0.5in,BUTTONHEAD,BOLT:16 ↔ PURCHASED,WASHER:12
- Insert:91: PLATE,HOOD,SIDE:2 ↔ PURCHASED,10-32x0.5in,BUTTONHEAD,BOLT:24
- Insert:92: PLATE,HOOD,SIDE:2 ↔ PURCHASED,10-32x0.5in,BUTTONHEAD,BOLT:25
- Insert:93: PLATE,HOOD,SIDE:2 ↔ PURCHASED,10-32x0.5in,BUTTONHEAD,BOLT:26
- Mate:120: PLATE,SHOOTER,SIDE:1 ↔ PLATE,SHOOTER,BOTTOM:1
- Mate:121: PURCHASED,HEX_BEARING:14 ↔ STOCK,SHAFT,HEX,HOOD,WHEELS,LONG:1
- Mate:122: PURCHASED,HEX_BEARING:14 ↔ STOCK,SHAFT,HEX,HOOD,WHEELS,LONG:1
- Insert:94: PLATE,BEARING,MOUNT:1 ↔ PURCHASED,HEX_BEARING:15
- Insert:96: PLATE,BEARING,MOUNT:1 ↔ PURCHASED,HEX_BEARING:14
- Mate:123: PURCHASED,HEX_BEARING:15 ↔ STOCK,SHAFT,HEX,HOOD,REVERSER:1
- Insert:97: PURCHASED,10-32,0.375inOD,STANDOFF:1 ↔ PLATE,BEARING,MOUNT:1
- Insert:98: PLATE,BEARING,MOUNT:1 ↔ PURCHASED,10-32x0.5in,BUTTONHEAD,BOLT:22
- Insert:99: PLATE,BEARING,MOUNT:1 ↔ PURCHASED,10-32x0.5in,BUTTONHEAD,BOLT:21
- Insert:100: PLATE,BEARING,MOUNT:1 ↔ PURCHASED,10-32x0.5in,BUTTONHEAD,BOLT:23
- Mate:124: STOCK,SHAFT,HEX,HOOD,REVERSER:1 ↔ PURCHASED,GEAR,20DP,30T,HEX:1
- Mate:125: STOCK,SHAFT,HEX,HOOD,REVERSER:1 ↔ PURCHASED,GEAR,20DP,30T,HEX:1
- Mate:126: STOCK,SHAFT,HEX,HOOD,WHEELS,LONG:1 ↔ PURCHASED,GEAR,20DP,30T,HEX:2
- Mate:127: STOCK,SHAFT,HEX,HOOD,WHEELS,LONG:1 ↔ PURCHASED,GEAR,20DP,30T,HEX:2
- Mate:128: PURCHASED,HEX_BEARING:7 ↔ PURCHASED,GEAR,20DP,30T,HEX:2
- Mate:129: PURCHASED,HEX_BEARING:12 ↔ PURCHASED,GEAR,20DP,30T,HEX:1
- Mate:131: PLATE,SHOOTER,BOTTOM:1 ↔ 3DPRINT,BACKRAIL:1
- Symmetry:1: PLATE,HOOD,SIDE:1 ↔ PLATE,HOOD,SIDE:2
- Insert:101: PLATE,SHOOTER,SIDE:2 ↔ PLATE,NUTBLOCK:1
- Insert:102: PLATE,SHOOTER,BOTTOM:1 ↔ PLATE,NUTBLOCK:1
- Insert:103: PLATE,SHOOTER,BOTTOM:1 ↔ PLATE,NUTBLOCK:2
- Insert:104: PLATE,SHOOTER,SIDE:2 ↔ PLATE,NUTBLOCK:2
- Insert:107: PLATE,SHOOTER,BOTTOM:1 ↔ PLATE,NUTBLOCK:4
- Insert:110: PLATE,SHOOTER,SIDE:1 ↔ PLATE,NUTBLOCK:5
- Insert:111: PLATE,SHOOTER,SIDE:1 ↔ PURCHASED,10-32x0.5in,BUTTONHEAD,BOLT:30
- Insert:112: PLATE,SHOOTER,SIDE:1 ↔ PURCHASED,10-32x0.5in,BUTTONHEAD,BOLT:29
- Insert:113: PLATE,SHOOTER,SIDE:1 ↔ PURCHASED,10-32x0.5in,BUTTONHEAD,BOLT:28
- Insert:114: PLATE,SHOOTER,SIDE:1 ↔ PURCHASED,10-32x0.5in,BUTTONHEAD,BOLT:27
- Insert:115: PLATE,SHOOTER,BOTTOM:1 ↔ PURCHASED,10-32x0.5in,BUTTONHEAD,BOLT:31
- Insert:116: PLATE,SHOOTER,BOTTOM:1 ↔ PURCHASED,10-32x0.5in,BUTTONHEAD,BOLT:32
- Insert:117: PLATE,SHOOTER,BOTTOM:1 ↔ PURCHASED,10-32x0.5in,BUTTONHEAD,BOLT:33
- Insert:118: PLATE,SHOOTER,BOTTOM:1 ↔ PURCHASED,10-32x0.5in,BUTTONHEAD,BOLT:34
- Insert:119: PLATE,SHOOTER,BOTTOM:1 ↔ PURCHASED,10-32x0.5in,BUTTONHEAD,BOLT:35
- Insert:120: PLATE,SHOOTER,BOTTOM:1 ↔ PURCHASED,10-32x0.5in,BUTTONHEAD,BOLT:36
- Insert:121: PLATE,SHOOTER,BOTTOM:1 ↔ PURCHASED,10-32x0.5in,BUTTONHEAD,BOLT:37
- Insert:122: PLATE,SHOOTER,BOTTOM:1 ↔ PURCHASED,10-32x0.5in,BUTTONHEAD,BOLT:38
- Insert:124: PLATE,SHOOTER,SIDE:2 ↔ PURCHASED,10-32x0.5in,BUTTONHEAD,BOLT:40
- Insert:125: PLATE,SHOOTER,SIDE:2 ↔ PURCHASED,10-32x0.5in,BUTTONHEAD,BOLT:41
- Insert:126: PLATE,SHOOTER,SIDE:2 ↔ PURCHASED,10-32x0.5in,BUTTONHEAD,BOLT:42
- Insert:127: PLATE,SHOOTER,SIDE:2 ↔ PURCHASED,10-32x0.5in,BUTTONHEAD,BOLT:43
- Insert:128: PLATE,SHOOTER,BACK:1 ↔ PURCHASED,10-32x0.5in,BUTTONHEAD,BOLT:44
- Insert:129: PLATE,SHOOTER,BACK:1 ↔ PURCHASED,10-32x0.5in,BUTTONHEAD,BOLT:45
- Insert:137: PLATE,SHOOTER,BOTTOM:1 ↔ PURCHASED,M4x12mm,BUTTONHEAD,BOLT:1
- Insert:138: PLATE,SHOOTER,BOTTOM:1 ↔ PURCHASED,M4x12mm,BUTTONHEAD,BOLT:2
- Insert:139: PLATE,SHOOTER,BOTTOM:1 ↔ PURCHASED,M4x12mm,BUTTONHEAD,BOLT:3
- Insert:140: PLATE,SHOOTER,BOTTOM:1 ↔ PURCHASED,M4x12mm,BUTTONHEAD,BOLT:4
- Insert:141: PLATE,SHOOTER,BOTTOM:1 ↔ PURCHASED,M4x12mm,BUTTONHEAD,BOLT:5
- Insert:142: PLATE,SHOOTER,BOTTOM:1 ↔ PURCHASED,M4x12mm,BUTTONHEAD,BOLT:6
- Insert:143: PLATE,SHOOTER,BOTTOM:1 ↔ PURCHASED,M4x12mm,BUTTONHEAD,BOLT:7
- Insert:144: PLATE,SHOOTER,BOTTOM:1 ↔ PURCHASED,M4x12mm,BUTTONHEAD,BOLT:8
- Insert:145: PLATE,SHOOTER,SIDE:2 ↔ PURCHASED,0.25-20x0.5in,BUTTONHEAD,BOLT:4
- Insert:146: PLATE,SHOOTER,SIDE:1 ↔ PURCHASED,0.25-20x0.5in,BUTTONHEAD,BOLT:1
- Insert:151: PLATE,SHOOTER,BOTTOM:1 ↔ 3DPRINT,BACKRAIL_MIR:1
- Mate:137: PLATE,SHOOTER,BOTTOM:1 ↔ 3DPRINT,BACKRAIL_MIR:1
- Mate:141: STOCK,SHAFT,HEX,SHOOTER:1 ↔ PURCHASED,HTD5mm,20T,PULLEY:3
- Mate:142: STOCK,SHAFT,HEX,SHOOTER:1 ↔ PURCHASED,HTD5mm,20T,PULLEY:3
- Mate:144: STOCK,SHAFT,HEX,HOOD,REVERSER:1 ↔ PURCHASED,HTD5mm,20T,PULLEY:4
- Mate:145: STOCK,SHAFT,HEX,HOOD,REVERSER:1 ↔ PURCHASED,HTD5mm,20T,PULLEY:4
- Mate:146: PURCHASED,GEAR,20DP,30T,HEX:1 ↔ PURCHASED,HTD5mm,20T,PULLEY:4
- Mate:147: PLATE,HOOD,SIDE:2 ↔ STANDIN,45T,HTD5mm,BELT:1
- Mate:148: PLATE,HOOD,SIDE:2 ↔ STANDIN,45T,HTD5mm,BELT:1
- Mate:149: PLATE,SHOOTER,SIDE:2 ↔ STANDIN,90T,HTD5mm,BELT:1
- Mate:150: PLATE,HOOD,SIDE:2 ↔ STANDIN,90T,HTD5mm,BELT:1
- Mate:151 (0.75 mm): PURCHASED,HTD5mm,20T,PULLEY:4 ↔ STANDIN,90T,HTD5mm,BELT:1
- Mate:152 (0.75 mm): PURCHASED,HTD5mm,20T,PULLEY:1 ↔ STANDIN,45T,HTD5mm,BELT:1
- Flush:9: STOCK,SHAFT,HEX,SHOOTER:1 ↔ PURCHASED,HTD5mm,20T,PULLEY:3
- Mate:153: STOCK,SHAFT,HEX,SHOOTER:1 ↔ 3DPRINT,FLYWHEELTOHOOD,SPACER:1
- Mate:154: STOCK,SHAFT,HEX,SHOOTER:1 ↔ 3DPRINT,FLYWHEELTOHOOD,SPACER:1
- Mate:155: PURCHASED,HEX_BEARING:9 ↔ 3DPRINT,FLYWHEELTOHOOD,SPACER:1
- Insert:152: PLATE,HOOD,SIDE:1 ↔ STOCK,HOOD,SPACER,10-32,6.25in:1
- Insert:153: PLATE,HOOD,SIDE:2 ↔ STOCK,HOOD,SPACER,10-32,6.25in:2
- Insert:154: PLATE,HOOD,SIDE:1 ↔ PURCHASED,10-32x0.5in,BUTTONHEAD,BOLT:49
- Insert:155: PLATE,HOOD,SIDE:1 ↔ PURCHASED,10-32x0.5in,BUTTONHEAD,BOLT:51
- Insert:156: PLATE,HOOD,SIDE:2 ↔ PURCHASED,10-32x0.5in,BUTTONHEAD,BOLT:50
- Insert:157: PLATE,HOOD,SIDE:2 ↔ PURCHASED,10-32x0.5in,BUTTONHEAD,BOLT:52
- Insert:158: PLATE,SHOOTER,BOTTOM:1 ↔ 3DPRINT,BACKRAIL:1
- Mate:157: STOCK,SHAFT,HEX,SHOOTER:1 ↔ 3DPRINT,SIDEPLATETOHOOD,SPACER :1
- Mate:158: STOCK,SHAFT,HEX,SHOOTER:1 ↔ 3DPRINT,SIDEPLATETOHOOD,SPACER :1
- Mate:159: PURCHASED,HEX_BEARING:11 ↔ 3DPRINT,SIDEPLATETOHOOD,SPACER :1
- Mate:160: STOCK,SHAFT,HEX,SHOOTER:1 ↔ 3DPRINT,SIDEPLATETOHOOD,SPACER :2
- Mate:161: STOCK,SHAFT,HEX,SHOOTER:1 ↔ 3DPRINT,SIDEPLATETOHOOD,SPACER :2
- Mate:162: PURCHASED,HEX_BEARING:10 ↔ 3DPRINT,SIDEPLATETOHOOD,SPACER :2
- Mate:163: PLATE.HOOD,PINION,GEAR:1 ↔ 3DPRINT,HOOD,DRIVEGEAR,SPACER:1
- Mate:164: STOCK,HEX,ROUND,HOOD:1 ↔ 3DPRINT,BUSHINGTOHOODDRIVEGEAR,SPACER:1
- Mate:165: STOCK,HEX,ROUND,HOOD:1 ↔ 3DPRINT,BUSHINGTOHOODDRIVEGEAR,SPACER:1
- Mate:166: PURCHASED,BUSHING,13.75mmID,0.75inOD:1 ↔ 3DPRINT,BUSHINGTOHOODDRIVEGEAR,SPACER:1
- Mate:167: PLATE.HOOD,PINION,GEAR:1 ↔ 3DPRINT,BUSHINGTOHOODDRIVEGEAR,SPACER:1
- Mate:168: STOCK,HEX,ROUND,HOOD:1 ↔ 3DPRINT,BUSHINGTOHOODDRIVEGEAR,SPACER:2
- Mate:169: STOCK,HEX,ROUND,HOOD:1 ↔ 3DPRINT,BUSHINGTOHOODDRIVEGEAR,SPACER:2
- Mate:170: PURCHASED,BUSHING,13.75mmID,0.75inOD:2 ↔ 3DPRINT,BUSHINGTOHOODDRIVEGEAR,SPACER:2
- Mate:171: STOCK,HEX,ROUND,HOOD:1 ↔ 3DPRINT,SIDEPLATETOHOODGEAR,SPACER:1
- Mate:172: STOCK,HEX,ROUND,HOOD:1 ↔ 3DPRINT,SIDEPLATETOHOODGEAR,SPACER:1
- Mate:173: PURCHASED,BUSHING,13.75mmID,0.75inOD:1 ↔ 3DPRINT,SIDEPLATETOHOODGEAR,SPACER:1
- Mate:174: PLATE,HOOD,SIDE:1 ↔ PLATE,SHOOTER,BOTTOM:1
- Insert:161: PLATE,HOOD,SIDE:1 ↔ 3DPRINT,HOOD,ALIGNMENT,PLATES:1
- Insert:163: PLATE,HOOD,SIDE:1 ↔ 3DPRINT,HOOD,ALIGNMENT,PLATES:2
- Insert:164: PLATE,HOOD,SIDE:1 ↔ 3DPRINT,HOOD,ALIGNMENT,PLATES:2
- Insert:165: PLATE,HOOD,SIDE:1 ↔ 3DPRINT,HOOD,ALIGNMENT,PLATES:1
- Insert:166: PLATE,HOOD,SIDE:2 ↔ 3DPRINT,HOOD,ALIGNMENT,PLATES:3
- Insert:167: PLATE,HOOD,SIDE:2 ↔ 3DPRINT,HOOD,ALIGNMENT,PLATES:3
- Insert:168: PLATE,HOOD,SIDE:2 ↔ 3DPRINT,HOOD,ALIGNMENT,PLATES:4
- Insert:169: PLATE,HOOD,SIDE:2 ↔ 3DPRINT,HOOD,ALIGNMENT,PLATES:4